# Autodesk Inventor assembly: controller
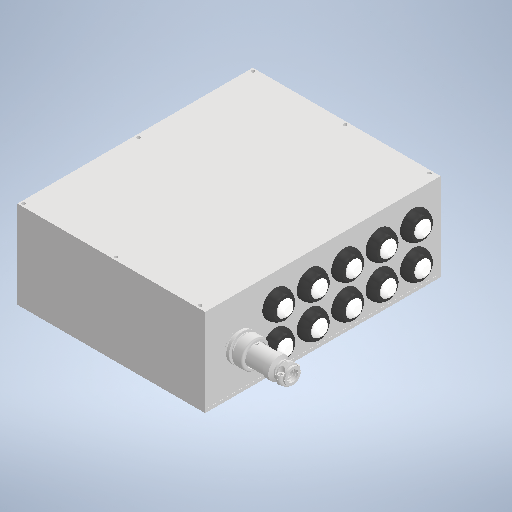
[picture p0: Inventor's stored thumbnail of the model, 512x512]
Saved by Autodesk Inventor 2025.2 (Build 292293000, 293)
## iProperties
Created: 2025-04-21
Part Number: controller
Document SubType Name: Assembly
Designer: tdeboutte
Author: tdeboutte
## Documents named in this file (6)
- C:\Users\tdeboutte\Documents\Projects\bluesmobile\CAD\controller.iam
- C:\Users\tdeboutte\Documents\Projects\bluesmobile\CAD\button-front.ipt
- C:\Users\tdeboutte\Documents\Projects\bluesmobile\CAD\controller-base.ipt
- C:\Users\tdeboutte\Documents\Projects\bluesmobile\CAD\controller-top.ipt
- C:\Users\tdeboutte\Documents\Projects\bluesmobile\CAD\Components\12mm Push Button Amazon\12mm Push Button Amazon.ipt
- C:\Users\tdeboutte\Documents\Projects\bluesmobile\CAD\Components\GX16-4P v2\GX16-4P v2.ipt
## Components (14 placed, 5 different names)
1. button-front:1 — Mate:1, Mate:2, Flush:1, Insert:1, Insert:2, Insert:3, Insert:4, Insert:5, Insert:6, Insert:7, Insert:8, Insert:9, Insert:10
2. controller-base:1 — Mate:1, Mate:2, Flush:1, Flush:2, Flush:3
3. controller-top:1 — Flush:2, Flush:3
4. 12mm Push Button Amazon:1 — Insert:3
5. 12mm Push Button Amazon:2 — Insert:6
6. 12mm Push Button Amazon:3 — Insert:5
7. 12mm Push Button Amazon:4 — Insert:7
8. 12mm Push Button Amazon:5 — Insert:9
9. 12mm Push Button Amazon:6 — Insert:10
10. 12mm Push Button Amazon:7 — Insert:8
11. 12mm Push Button Amazon:8 — Insert:2
12. 12mm Push Button Amazon:9 — Insert:1
13. 12mm Push Button Amazon:10 — Insert:4
14. GX16-4P v2:1
## Relationships (16: Insert 11, Flush 3, Mate 2)
- Mate:1: button-front:1 ↔ controller-base:1
- Mate:2: button-front:1 ↔ controller-base:1
- Flush:1: button-front:1 ↔ controller-base:1
- Flush:2: controller-base:1 ↔ controller-top:1
- Flush:3: controller-base:1 ↔ controller-top:1
- Insert:1: button-front:1 ↔ 12mm Push Button Amazon:9
- Insert:2: button-front:1 ↔ 12mm Push Button Amazon:8
- Insert:3: button-front:1 ↔ 12mm Push Button Amazon:1
- Insert:4: button-front:1 ↔ 12mm Push Button Amazon:10
- Insert:5: button-front:1 ↔ 12mm Push Button Amazon:3
- Insert:6: button-front:1 ↔ 12mm Push Button Amazon:2
- Insert:7: button-front:1 ↔ 12mm Push Button Amazon:4
- Insert:8: button-front:1 ↔ 12mm Push Button Amazon:7
- Insert:9: button-front:1 ↔ 12mm Push Button Amazon:5
- Insert:10: button-front:1 ↔ 12mm Push Button Amazon:6
- [Insert]: button-front:1 ↔ GX16-4P v2:1
## Named parameters: d16_d0 = 0 mm
